# Autodesk Inventor assembly: Link_02_Assembly_V02
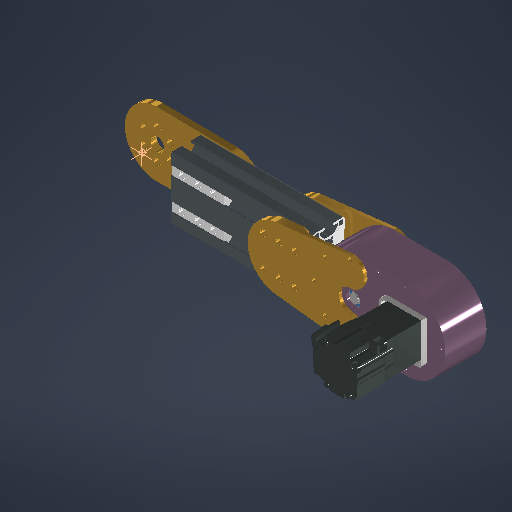
[picture p0: Inventor's stored thumbnail of the model, 512x512]
Saved by Autodesk Inventor 2026 (Build 300175000, 175)
## iProperties
Created: 2025-12-01
Part Number: Link_02_Assembly_V02
Document SubType Name: Assembly
Designer: DanielFGarzon
Mass: 1472.35 g
Surface Area: 2661.67 cm^2
Volume: 491.537 cm^3
Density: 2.99539 g/cm^3
Author: DanielFGarzon
## Documents named in this file (5)
- D:\POLIMI\3RD SEMESTER\Industrial Robotics\Project\Mine\Inventor_Files\Link_02_Assembly_V04.iam
- D:\POLIMI\3RD SEMESTER\Industrial Robotics\Project\Mine\Inventor_Files\Link_02_V03.ipt
- D:\POLIMI\3RD SEMESTER\Industrial Robotics\Project\Mine\Inventor_Files\Reducer_02\Reducer_Motor_HG-KR53.iam
- D:\POLIMI\3RD SEMESTER\Industrial Robotics\Project\Mine\Inventor_Files\Reducer_02\RigidConector_30x60_v04.ipt
- D:\POLIMI\3RD SEMESTER\Industrial Robotics\Project\Mine\Inventor_Files\Reducer_02\RotationalConector_30x60_V04.ipt
## Components (5 placed, 4 different names)
1. Link_02_V03:1 — Mate:16, Flush:1, Mate:17, Mate:18, Mate:19, Mate:20, Mate:21, Mate:22, Mate:27, Mate:28, Mate:29
2. RotationalConector_30x60_V04:1 — Mate:26, Mate:27, Mate:28, Mate:29
3. Reducer_Motor_HG-KR53:1 [sub-assembly] — Mate:23, Mate:24, Mate:25
4. RigidConector_30x60_v04:1 — Mate:17, Mate:18, Mate:19, Mate:23, Mate:24, Mate:25
5. RigidConector_30x60_v04:2 — Mate:20, Mate:21, Mate:22
## Relationships (15: Mate 14, Flush 1)
- Mate:16: Link_02_V03:1
- Flush:1: Link_02_V03:1
- Mate:17: Link_02_V03:1 ↔ RigidConector_30x60_v04:1
- Mate:18: Link_02_V03:1 ↔ RigidConector_30x60_v04:1
- Mate:19: Link_02_V03:1 ↔ RigidConector_30x60_v04:1
- Mate:20: Link_02_V03:1 ↔ RigidConector_30x60_v04:2
- Mate:21: Link_02_V03:1 ↔ RigidConector_30x60_v04:2
- Mate:22: Link_02_V03:1 ↔ RigidConector_30x60_v04:2
- Mate:23: Reducer_Motor_HG-KR53:1 ↔ RigidConector_30x60_v04:1
- Mate:24: Reducer_Motor_HG-KR53:1 ↔ RigidConector_30x60_v04:1
- Mate:25: Reducer_Motor_HG-KR53:1 ↔ RigidConector_30x60_v04:1
- Mate:26: RotationalConector_30x60_V04:1
- Mate:27: Link_02_V03:1 ↔ RotationalConector_30x60_V04:1
- Mate:28: Link_02_V03:1 ↔ RotationalConector_30x60_V04:1
- Mate:29: Link_02_V03:1 ↔ RotationalConector_30x60_V04:1
